# Autodesk Inventor assembly: test2
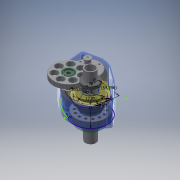
[picture p0: Inventor's stored thumbnail of the model, 180x180]
Saved by Autodesk Inventor 2018.1 (Build 221171000, 171)
## iProperties
Created: 2022-07-20
Part Number: test2
Document SubType Name: Assembly
Designer: mouta
Author: mouta
## Documents named in this file (4)
- C:\Users\Bureau\Mon Drive\Manu\USINAGE\MoteurVelo\test2.iam
- C:\Users\Bureau\Mon Drive\Manu\USINAGE\MoteurVelo\Corps\body depart.ipt
- C:\Users\Bureau\Mon Drive\Manu\USINAGE\MoteurVelo\Assembly4.iam
- C:\Users\Bureau\Mon Drive\Manu\USINAGE\MoteurVelo\Corps\body cote droit.ipt
## Components (3 placed, 3 different names)
1. body depart:1 — Mate:2, Flush:2, Mate:4
2. Assembly4:1 [sub-assembly] — Mate:2, Flush:2, Mate:3
3. body cote droit:1 — Mate:3, Mate:4
## Relationships (4: Mate 3, Flush 1)
- Mate:2: body depart:1 ↔ Assembly4:1
- Flush:2 (50 mm): body depart:1 ↔ Assembly4:1
- Mate:3: Assembly4:1 ↔ body cote droit:1
- Mate:4: body depart:1 ↔ body cote droit:1
